# Autodesk Inventor assembly: Hanabi
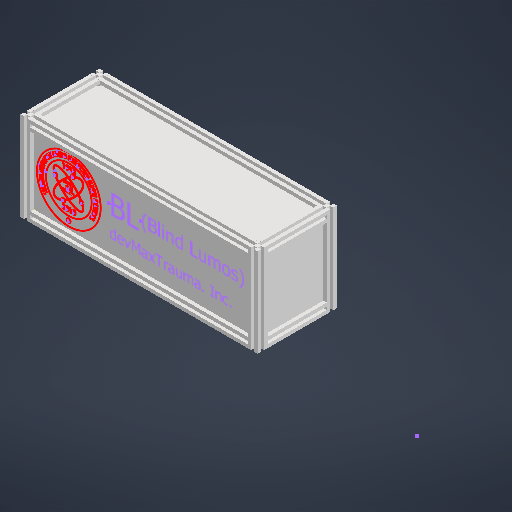
[picture p0: Inventor's stored thumbnail of the model, 512x512]
Saved by Autodesk Inventor 2025.1 (Build 291241020, 241B)
## iProperties
Created: 2024-09-23
Part Number: Hanabi
Document SubType Name: Assembly
Designer: techn
Author: techn
## Documents named in this file (8)
- C:\Users\techn\OneDrive\devMaxTrauma\3DModel\Hanabi.iam
- C:\Users\techn\OneDrive\devMaxTrauma\3DModel\hanabi plate.ipt
- C:\Users\techn\OneDrive\devMaxTrauma\3DModel\xbar.ipt
- C:\Users\techn\OneDrive\devMaxTrauma\3DModel\ybar.ipt
- C:\Users\techn\OneDrive\devMaxTrauma\3DModel\zbar.ipt
- C:\Users\techn\OneDrive\devMaxTrauma\3DModel\zpanel.ipt
- C:\Users\techn\OneDrive\devMaxTrauma\3DModel\ypanel.ipt
- C:\Users\techn\OneDrive\devMaxTrauma\3DModel\xpanel.ipt
## Components (18 placed, 7 different names)
1. hanabi plate:1 — Flush:1, Flush:2
2. xbar:1 — Flush:1, Rigid:1, Rigid:2
3. xbar:2 — Rigid:1
4. ybar:1 — Flush:2, Rigid:4, Rigid:5
5. ybar:2 — Rigid:2, Flush:3, Rigid:3
6. zbar:1 — Flush:3
7. zbar:2 — Rigid:5, Rigid:7
8. zbar:3 — Rigid:4, Flush:5
9. zbar:4 — Rigid:3, Rigid:6
10. ybar:3 — Rigid:7, Rigid:8, Flush:6
11. ybar:4 — Rigid:6, Rigid:9, Flush:4
12. xbar:3 — Rigid:8
13. xbar:4 — Rigid:9
14. zpanel:1 — Flush:4
15. ypanel:1 — Flush:5, Rigid:10
16. ypanel:2 — Rigid:10
17. xpanel:1 — Flush:6, Rigid:11
18. xpanel:2 — Rigid:11
## Relationships (17: WeldJoint 11, Flush 6)
- Flush:1 (-5 mm): hanabi plate:1 ↔ xbar:1
- Rigid:1 [WeldJoint] (-140 mm): xbar:1 ↔ xbar:2
- Flush:2: hanabi plate:1 ↔ ybar:1
- Rigid:2 [WeldJoint]: xbar:1 ↔ ybar:2
- Flush:3: ybar:2 ↔ zbar:1
- Rigid:3 [WeldJoint]: ybar:2 ↔ zbar:4
- Rigid:4 [WeldJoint]: ybar:1 ↔ zbar:3
- Rigid:5 [WeldJoint]: ybar:1 ↔ zbar:2
- Rigid:6 [WeldJoint]: zbar:4 ↔ ybar:4
- Rigid:7 [WeldJoint]: zbar:2 ↔ ybar:3
- Rigid:8 [WeldJoint]: ybar:3 ↔ xbar:3
- Rigid:9 [WeldJoint]: ybar:4 ↔ xbar:4
- Flush:4: ybar:4 ↔ zpanel:1
- Flush:5: zbar:3 ↔ ypanel:1
- Rigid:10 [WeldJoint] (-155 mm): ypanel:1 ↔ ypanel:2
- Flush:6: ybar:3 ↔ xpanel:1
- Rigid:11 [WeldJoint] (-460 mm): xpanel:1 ↔ xpanel:2
